# Autodesk Inventor assembly: Xaxis
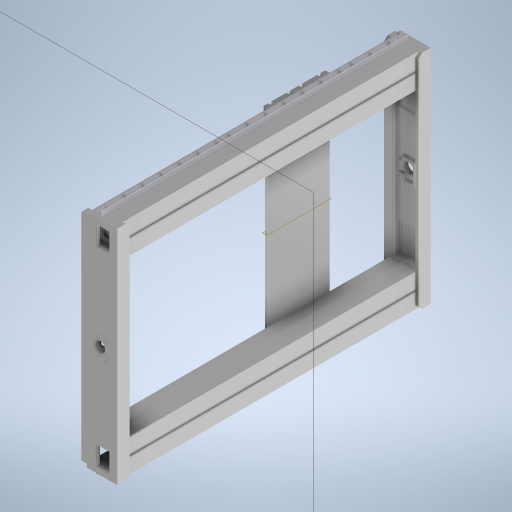
[picture p0: Inventor's stored thumbnail of the model, 512x512]
Saved by Autodesk Inventor 2024 (Build 280153000, 153)
## iProperties
Created: 2023-03-08
Part Number: Xaxis
Document SubType Name: Assembly
Designer: KirikDK
Author: KirikDK
## Documents named in this file (4)
- C:\Users\KirikDK\Documents\Stanok2023\Xaxis.iam
- C:\Users\KirikDK\Documents\Stanok2023\FlanecX_Aax.ipt
- C:\Users\KirikDK\Documents\Stanok2023\RailBlock.iam
- C:\Users\KirikDK\Documents\Stanok2023\TopPaz.ipt
## Components (6 placed, 3 different names)
1. FlanecX_Aax:1 — Совмещение:1, Совмещение:2, Заподлицо:1, Совмещение:3, Совмещение:4, Заподлицо:2
2. RailBlock:2 [sub-assembly] — Совмещение:1, Совмещение:2, Заподлицо:1
3. RailBlock:3 [sub-assembly] — Совмещение:3, Совмещение:4, Заподлицо:2, Совмещение:5, Совмещение:6, Заподлицо:3, Совмещение:7, Заподлицо:4, Заподлицо:5, Совмещение:8
4. FlanecX_Aax:2 — Совмещение:5, Совмещение:6, Заподлицо:3
5. TopPaz:1 — Совмещение:7, Заподлицо:4, Совмещение:9
6. TopPaz:2 — Заподлицо:5, Совмещение:8, Совмещение:9
## Relationships (14: Mate 9, Flush 5)
- Совмещение:1 [Mate]: FlanecX_Aax:1 ↔ RailBlock:2
- Совмещение:2 [Mate]: FlanecX_Aax:1 ↔ RailBlock:2
- Заподлицо:1 [Flush]: FlanecX_Aax:1 ↔ RailBlock:2
- Совмещение:3 [Mate]: FlanecX_Aax:1 ↔ RailBlock:3
- Совмещение:4 [Mate]: FlanecX_Aax:1 ↔ RailBlock:3
- Заподлицо:2 [Flush]: FlanecX_Aax:1 ↔ RailBlock:3
- Совмещение:5 [Mate]: RailBlock:3 ↔ FlanecX_Aax:2
- Совмещение:6 [Mate]: RailBlock:3 ↔ FlanecX_Aax:2
- Заподлицо:3 [Flush]: RailBlock:3 ↔ FlanecX_Aax:2
- Совмещение:7 [Mate]: RailBlock:3 ↔ TopPaz:1
- Заподлицо:4 [Flush]: RailBlock:3 ↔ TopPaz:1
- Заподлицо:5 [Flush]: RailBlock:3 ↔ TopPaz:2
- Совмещение:8 [Mate]: RailBlock:3 ↔ TopPaz:2
- Совмещение:9 [Mate]: TopPaz:1 ↔ TopPaz:2
